# Autodesk Inventor assembly: Assembly1
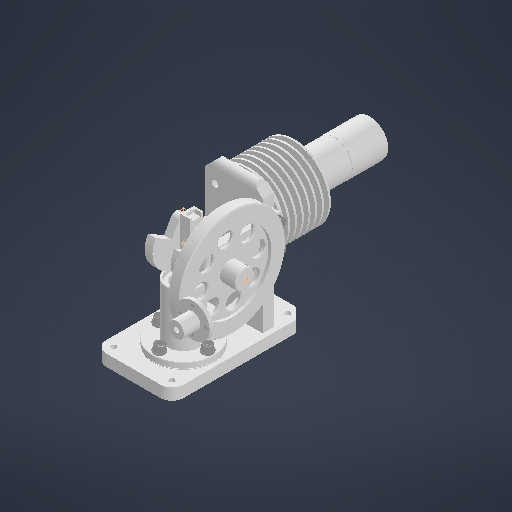
[picture p0: Inventor's stored thumbnail of the model, 512x512]
Saved by Autodesk Inventor 2025.4 (Build 294407000, 407)
## iProperties
Created: 2026-06-01
Part Number: Assembly1
Document SubType Name: Assembly
Designer: VuQuan
Author: VuQuan
## Documents named in this file (30)
- D:\Edu\4CHaUI-Inventor\Assembly\b2\Assembly1.iam
- D:\Edu\4CHaUI-Inventor\Assembly\b2\Base.ipt
- D:\Edu\4CHaUI-Inventor\Assembly\b2\Cylinder.ipt
- D:\Edu\4CHaUI-Inventor\Assembly\b2\CylinderPacking.ipt
- D:\Edu\4CHaUI-Inventor\Assembly\b2\Standard.ipt
- D:\Edu\4CHaUI-Inventor\Assembly\b2\Support.ipt
- D:\Edu\4CHaUI-Inventor\Assembly\b2\DIN 912 - M6 x 1 x 20 x 17.5.ipt
- D:\Edu\4CHaUI-Inventor\Assembly\b2\ISO 8734 - 5 x 20 - AISO (1).ipt
- D:\Edu\4CHaUI-Inventor\Assembly\b2\ISO 8734 - 3 x 16 - AISO (1).ipt
- D:\Edu\4CHaUI-Inventor\Assembly\b2\DIN 912 - M6 x 1 x 16 x 13.5.ipt
- D:\Edu\4CHaUI-Inventor\Assembly\b2\HeatExchangeCylinder.ipt
- D:\Edu\4CHaUI-Inventor\Assembly\b2\HeatExchangeCylinderhead.ipt
- D:\Edu\4CHaUI-Inventor\Assembly\b2\HeatExchangePistonExhaust.ipt
- D:\Edu\4CHaUI-Inventor\Assembly\b2\HeatExchangePistonHead.ipt
- D:\Edu\4CHaUI-Inventor\Assembly\b2\HeatExchangePistonShaft.ipt
- D:\Edu\4CHaUI-Inventor\Assembly\b2\HeatExchangePistonTube.ipt
- D:\Edu\4CHaUI-Inventor\Assembly\b2\BearingSuport.ipt
- D:\Edu\4CHaUI-Inventor\Assembly\b2\CounterweightA.ipt
- D:\Edu\4CHaUI-Inventor\Assembly\b2\CounterweightB.ipt
- D:\Edu\4CHaUI-Inventor\Assembly\b2\Crankrod.ipt
- D:\Edu\4CHaUI-Inventor\Assembly\b2\CrankShaft.ipt
- D:\Edu\4CHaUI-Inventor\Assembly\b2\Crosshead.ipt
- D:\Edu\4CHaUI-Inventor\Assembly\b2\Flywheel.ipt
- D:\Edu\4CHaUI-Inventor\Assembly\b2\Flywheelshaft.ipt
- D:\Edu\4CHaUI-Inventor\Assembly\b2\Piston.ipt
- D:\Edu\4CHaUI-Inventor\Assembly\b2\PistonPin.ipt
- D:\Edu\4CHaUI-Inventor\Assembly\b2\Slide.ipt
- D:\Edu\4CHaUI-Inventor\Assembly\b2\DIN 913 - M5 x 8.ipt
- D:\Edu\4CHaUI-Inventor\Assembly\b2\DIN 128 - A6.ipt
- D:\Edu\4CHaUI-Inventor\Assembly\b2\DIN 912 - M6 x 1 x 20 x 17.5 (1).ipt
## Components (39 placed, 29 different names)
1. Base:1 — Insert:3, Insert:4, Insert:5, Insert:6, Mate:3, Insert:19, Mate:4, Mate:5, Mate:6, Tangent:1, Tangent:2
2. Cylinder:1 — Insert:7, Insert:8, Insert:9, Insert:10, Insert:11, Insert:12, Mate:18
3. CylinderPacking:1 — Insert:5, Insert:6, Insert:7, Insert:8
4. Standard:1 — Mate:1, Mate:2, Insert:1, Insert:2, Insert:3, Insert:4, Insert:22, Insert:23
5. Support:1 — Insert:1, Insert:2, Insert:17, Insert:18, Mate:7, Mate:8, Tangent:3, Tangent:4, Mate:21
6. DIN 912 - M6 x 1 x 20 x 17.5:1 — Insert:18
7. DIN 912 - M6 x 1 x 20 x 17.5:2 — Insert:17
8. ISO 8734 - 5 x 20 - AISO (1):1 — Mate:6, Tangent:2
9. ISO 8734 - 5 x 20 - AISO (1):2 — Mate:5, Tangent:1
10. ISO 8734 - 3 x 16 - AISO (1):1 — Mate:7, Tangent:4
11. ISO 8734 - 3 x 16 - AISO (1):2 — Mate:8, Tangent:3
12. DIN 128 - A6:1 — Insert:9, Insert:16
13. DIN 128 - A6:2 — Insert:12, Insert:14
14. DIN 128 - A6:3 — Insert:10, Insert:13
15. DIN 128 - A6:4 — Insert:11, Insert:15
16. DIN 912 - M6 x 1 x 16 x 13.5:1 — Insert:13
17. DIN 912 - M6 x 1 x 16 x 13.5:2 — Insert:16
18. DIN 912 - M6 x 1 x 16 x 13.5:3 — Insert:15
19. DIN 912 - M6 x 1 x 16 x 13.5:4 — Insert:14
20. DIN 912 - M6 x 1 x 20 x 17.5 (1):1 — Mate:4
21. DIN 912 - M6 x 1 x 20 x 17.5 (1):2 — Insert:19
22. HeatExchangeCylinder:1 — Insert:20, Insert:22, Insert:23, Mate:11
23. HeatExchangeCylinderhead:1 — Insert:20
24. HeatExchangePistonExhaust:1 — Insert:24, Insert:25
25. HeatExchangePistonHead:1 — Insert:21
26. HeatExchangePistonShaft:1 — Insert:24, Insert:26, Mate:12
27. HeatExchangePistonTube:1 — Insert:21, Mate:11, Insert:25
28. BearingSuport:1
29. CounterweightA:1 — Angle:2, Insert:28, Insert:30
30. CounterweightB:1 — Angle:2, Insert:27
31. Crankrod:1 — Mate:19, Mate:24
32. CrankShaft:1 — Mate:20, Insert:27, Insert:28, Mate:24
33. Crosshead:1 — Insert:26, Mate:13, Angle:1, Mate:22, Mate:23
34. Flywheel:1 — Insert:29
35. Flywheelshaft:1 — Insert:29, Mate:21, Insert:30
36. Piston:1 — Mate:17, Tangent:5, Mate:18
37. PistonPin:1 — Mate:17, Tangent:5, Mate:19
38. Slide:1 — Mate:20, Mate:22, Mate:23
39. DIN 913 - M5 x 8:1 — Mate:12, Mate:13
## Relationships (56: Insert 30, Mate 19, Tangent 5, Angle 2)
- Mate:1: Standard:1
- Mate:2: Standard:1
- Insert:1: Standard:1 ↔ Support:1
- Insert:2: Standard:1 ↔ Support:1
- Insert:3: Base:1 ↔ Standard:1
- Insert:4: Base:1 ↔ Standard:1
- Insert:5: Base:1 ↔ CylinderPacking:1
- Insert:6: Base:1 ↔ CylinderPacking:1
- Insert:7: Cylinder:1 ↔ CylinderPacking:1
- Mate:3: Base:1
- Insert:8: Cylinder:1 ↔ CylinderPacking:1
- Insert:9: Cylinder:1 ↔ DIN 128 - A6:1
- Insert:10: Cylinder:1 ↔ DIN 128 - A6:3
- Insert:11: Cylinder:1 ↔ DIN 128 - A6:4
- Insert:12: Cylinder:1 ↔ DIN 128 - A6:2
- Insert:13: DIN 128 - A6:3 ↔ DIN 912 - M6 x 1 x 16 x 13.5:1
- Insert:14: DIN 128 - A6:2 ↔ DIN 912 - M6 x 1 x 16 x 13.5:4
- Insert:15: DIN 128 - A6:4 ↔ DIN 912 - M6 x 1 x 16 x 13.5:3
- Insert:16: DIN 128 - A6:1 ↔ DIN 912 - M6 x 1 x 16 x 13.5:2
- Insert:17: Support:1 ↔ DIN 912 - M6 x 1 x 20 x 17.5:2
- Insert:18: Support:1 ↔ DIN 912 - M6 x 1 x 20 x 17.5:1
- Insert:19: Base:1 ↔ DIN 912 - M6 x 1 x 20 x 17.5 (1):2
- Mate:4: Base:1 ↔ DIN 912 - M6 x 1 x 20 x 17.5 (1):1
- Mate:5: Base:1 ↔ ISO 8734 - 5 x 20 - AISO (1):2
- Mate:6: Base:1 ↔ ISO 8734 - 5 x 20 - AISO (1):1
- Tangent:1: Base:1 ↔ ISO 8734 - 5 x 20 - AISO (1):2
- Tangent:2: Base:1 ↔ ISO 8734 - 5 x 20 - AISO (1):1
- Mate:7: Support:1 ↔ ISO 8734 - 3 x 16 - AISO (1):1
- Mate:8: Support:1 ↔ ISO 8734 - 3 x 16 - AISO (1):2
- Tangent:3: Support:1 ↔ ISO 8734 - 3 x 16 - AISO (1):2
- Tangent:4: Support:1 ↔ ISO 8734 - 3 x 16 - AISO (1):1
- Insert:20: HeatExchangeCylinder:1 ↔ HeatExchangeCylinderhead:1
- Insert:21: HeatExchangePistonHead:1 ↔ HeatExchangePistonTube:1
- Insert:22: Standard:1 ↔ HeatExchangeCylinder:1
- Insert:23: Standard:1 ↔ HeatExchangeCylinder:1
- Mate:11: HeatExchangeCylinder:1 ↔ HeatExchangePistonTube:1
- Insert:24: HeatExchangePistonExhaust:1 ↔ HeatExchangePistonShaft:1
- Insert:25: HeatExchangePistonExhaust:1 ↔ HeatExchangePistonTube:1
- Insert:26: HeatExchangePistonShaft:1 ↔ Crosshead:1
- Mate:12: HeatExchangePistonShaft:1 ↔ DIN 913 - M5 x 8:1
- Mate:13: Crosshead:1 ↔ DIN 913 - M5 x 8:1
- Angle:1 (180 deg): Crosshead:1
- Angle:2 (0 deg): CounterweightA:1 ↔ CounterweightB:1
- Mate:17: Piston:1 ↔ PistonPin:1
- Tangent:5: Piston:1 ↔ PistonPin:1
- Mate:18: Cylinder:1 ↔ Piston:1
- Mate:19: Crankrod:1 ↔ PistonPin:1
- Mate:20: CrankShaft:1 ↔ Slide:1
- Insert:27: CounterweightB:1 ↔ CrankShaft:1
- Insert:28: CounterweightA:1 ↔ CrankShaft:1
- Insert:29: Flywheel:1 ↔ Flywheelshaft:1
- Mate:21: Support:1 ↔ Flywheelshaft:1
- Insert:30: CounterweightA:1 ↔ Flywheelshaft:1
- Mate:22: Crosshead:1 ↔ Slide:1
- Mate:23: Crosshead:1 ↔ Slide:1
- Mate:24: Crankrod:1 ↔ CrankShaft:1
